# Autodesk Inventor assembly: licht_150_links
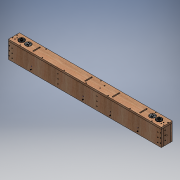
[picture p0: Inventor's stored thumbnail of the model, 180x180]
Saved by Autodesk Inventor 2016 SP2 (Build 200236200, 236)
## iProperties
Created: 2018-02-17
Part Number: licht_150_links
Document SubType Name: Assembly
Designer: wepet
Mass: 9428.77 g
Surface Area: 14177.6 cm^2
Volume: 9428.77 cm^3
Density: 1 g/cm^3
Author: wepet
## Documents named in this file (13)
- L:\Granz\RoboSAX\licht_150.iam
- L:\Granz\RoboSAX\licht_150_back.ipt
- L:\Granz\RoboSAX\licht_150_front.ipt
- L:\Granz\RoboSAX\licht_150_top.ipt
- L:\Granz\RoboSAX\licht_150_side_middle.ipt
- L:\Granz\RoboSAX\licht_led_blau.ipt
- L:\Granz\RoboSAX\licht_taster.ipt
- L:\Granz\RoboSAX\anschluss_strom.ipt
- L:\Granz\RoboSAX\anschluss_daten.iam
- L:\Granz\RoboSAX\licht_150_side_right.ipt
- L:\Granz\RoboSAX\licht_150_side_left.ipt
- L:\Granz\RoboSAX\licht_150_support_right.ipt
- L:\Granz\RoboSAX\licht_150_support_left.ipt
## Components (20 placed, 12 different names)
1. licht_led_blau:1 — Einfügen:4
2. licht_led_blau:2 — Einfügen:3
3. licht_led_blau:3 — Einfügen:1
4. licht_led_blau:4 — Einfügen:2
5. licht_taster:1 — Einfügen:5
6. licht_taster:2 — Einfügen:6
7. licht_taster:3 — Einfügen:7
8. licht_taster:4 — Einfügen:8
9. anschluss_strom:1 — Drehbar:1, Passend:26
10. anschluss_strom:2 — Passend:30, Passend:31, Passend:47
11. anschluss_daten:1 [sub-assembly] — Passend:27, Passend:28, Passend:29
12. anschluss_daten:2 [sub-assembly] — Passend:32, Passend:33, Passend:34
13. licht_150_front:1 — Passend:1, Passend:2, Passend:3, Passend:4, Fluchtend:1, Fluchtend:2, Fluchtend:3, Fluchtend:4, Einfügen:1, Einfügen:2, Einfügen:3, Einfügen:4, Einfügen:5, Einfügen:6, Einfügen:7, Einfügen:8, Passend:36, Passend:37, Fluchtend:12, Passend:39, Passend:42, Passend:45
14. licht_150_back:1 — Fluchtend:3, Fluchtend:4, Fluchtend:5, Passend:9, Fluchtend:13
15. licht_150_top:1 — Passend:4, Fluchtend:1, Fluchtend:2, Fluchtend:5, Passend:8, Drehbar:1, Passend:26, Passend:27, Passend:28, Passend:29, Passend:30, Passend:31, Passend:32, Passend:33, Passend:34, Passend:38, Passend:40, Passend:41, Passend:44, Passend:47
16. licht_150_side_right:1 — Passend:37, Fluchtend:12, Passend:38, Passend:43
17. licht_150_side_middle:1 — Passend:8, Passend:9, Passend:36
18. licht_150_side_left:1 — Passend:39, Passend:40, Fluchtend:13, Passend:46
19. licht_150_support_right:1 — Passend:41, Passend:42, Passend:43
20. licht_150_support_left:1 — Passend:44, Passend:45, Passend:46
## Relationships (43: Mate 27, Insert 8, Flush 7, RevoluteJoint 1)
- Passend:1 [Mate]: licht_150_front:1
- Passend:2 [Mate]: licht_150_front:1
- Passend:3 [Mate]: licht_150_front:1
- Passend:4 [Mate]: licht_150_front:1 ↔ licht_150_top:1
- Fluchtend:1 [Flush]: licht_150_front:1 ↔ licht_150_top:1
- Fluchtend:2 [Flush]: licht_150_front:1 ↔ licht_150_top:1
- Fluchtend:3 [Flush]: licht_150_front:1 ↔ licht_150_back:1
- Fluchtend:4 [Flush]: licht_150_front:1 ↔ licht_150_back:1
- Fluchtend:5 [Flush]: licht_150_back:1 ↔ licht_150_top:1
- Passend:8 [Mate]: licht_150_top:1 ↔ licht_150_side_middle:1
- Passend:9 [Mate]: licht_150_back:1 ↔ licht_150_side_middle:1
- Einfügen:1 [Insert] (-5 mm): licht_led_blau:3 ↔ licht_150_front:1
- Einfügen:2 [Insert] (-5 mm): licht_led_blau:4 ↔ licht_150_front:1
- Einfügen:3 [Insert]: licht_led_blau:2 ↔ licht_150_front:1
- Einfügen:4 [Insert]: licht_led_blau:1 ↔ licht_150_front:1
- Einfügen:5 [Insert] (5 mm): licht_taster:1 ↔ licht_150_front:1
- Einfügen:6 [Insert] (5 mm): licht_taster:2 ↔ licht_150_front:1
- Einfügen:7 [Insert] (5 mm): licht_taster:3 ↔ licht_150_front:1
- Einfügen:8 [Insert] (5 mm): licht_taster:4 ↔ licht_150_front:1
- Drehbar:1 [RevoluteJoint] (-7 mm): anschluss_strom:1 ↔ licht_150_top:1
- Passend:26 [Mate]: anschluss_strom:1 ↔ licht_150_top:1
- Passend:27 [Mate]: anschluss_daten:1 ↔ licht_150_top:1
- Passend:28 [Mate]: anschluss_daten:1 ↔ licht_150_top:1
- Passend:29 [Mate]: anschluss_daten:1 ↔ licht_150_top:1
- Passend:30 [Mate]: anschluss_strom:2 ↔ licht_150_top:1
- Passend:31 [Mate]: anschluss_strom:2 ↔ licht_150_top:1
- Passend:32 [Mate]: anschluss_daten:2 ↔ licht_150_top:1
- Passend:33 [Mate]: anschluss_daten:2 ↔ licht_150_top:1
- Passend:34 [Mate]: anschluss_daten:2 ↔ licht_150_top:1
- Passend:36 [Mate]: licht_150_front:1 ↔ licht_150_side_middle:1
- Passend:37 [Mate]: licht_150_front:1 ↔ licht_150_side_right:1
- Fluchtend:12 [Flush]: licht_150_front:1 ↔ licht_150_side_right:1
- Passend:38 [Mate]: licht_150_top:1 ↔ licht_150_side_right:1
- Passend:39 [Mate]: licht_150_front:1 ↔ licht_150_side_left:1
- Passend:40 [Mate]: licht_150_top:1 ↔ licht_150_side_left:1
- Fluchtend:13 [Flush]: licht_150_back:1 ↔ licht_150_side_left:1
- Passend:41 [Mate]: licht_150_top:1 ↔ licht_150_support_right:1
- Passend:42 [Mate]: licht_150_front:1 ↔ licht_150_support_right:1
- Passend:43 [Mate]: licht_150_side_right:1 ↔ licht_150_support_right:1
- Passend:44 [Mate]: licht_150_top:1 ↔ licht_150_support_left:1
- Passend:45 [Mate]: licht_150_front:1 ↔ licht_150_support_left:1
- Passend:46 [Mate]: licht_150_side_left:1 ↔ licht_150_support_left:1
- Passend:47 [Mate]: anschluss_strom:2 ↔ licht_150_top:1
